# Autodesk Inventor assembly: BaseBotNoMod
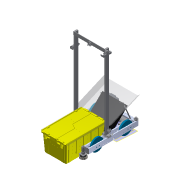
[picture p0: Inventor's stored thumbnail of the model, 180x180]
Saved by Autodesk Inventor 2015 (Build 190159000, 159)
## iProperties
Created: 2015-03-06
Part Number: BaseBotNoMod
Document SubType Name: Assembly
Designer: Kyle
Title: AM14U2 Long FIXED.STEP
Description: STEP AP214
Creation Date: 2015-01-13
Sending System: SolidWorks 2014
Preprocessor: SwSTEP 2.0
Author: Kyle
## Documents named in this file (29)
- C:\Users\Jaden\Desktop\This is why i dont sleep\2015CAD\ReDesign\Project.iam
- C:\Users\Jaden\Desktop\This is why i dont sleep\2015CAD\ReDesign\Imported Components\AM14U2+Long+FIXED\AM14U2 Half Long.iam
- C:\Users\Jaden\Desktop\This is why i dont sleep\2015CAD\ReDesign\Wheel.ipt
- C:\Users\Jaden\Desktop\This is why i dont sleep\2015CAD\ReDesign\Toughbox+Nano+All+Shafts+v2.iam
- C:\Users\Jaden\Desktop\This is why i dont sleep\2015CAD\ReDesign\ControlBoard.ipt
- C:\Users\Jaden\Desktop\This is why i dont sleep\2015CAD\ReDesign\LoadSlide.ipt
- C:\Users\Jaden\Desktop\This is why i dont sleep\2015CAD\ReDesign\FrontSet.ipt
- C:\Users\Jaden\Desktop\This is why i dont sleep\2015CAD\ReDesign\PEG.iam
- C:\Users\Jaden\Desktop\This is why i dont sleep\2015CAD\ReDesign\Slidev2.ipt
- C:\Users\Jaden\Desktop\This is why i dont sleep\2015CAD\ReDesign\YELLOW_TOTEASM_ASM.iam
- C:\Users\Jaden\Desktop\This is why i dont sleep\2015CAD\ReDesign\1x1tbar.ipt
- C:\Users\Jaden\Desktop\This is why i dont sleep\2015CAD\ReDesign\Lift Towers.ipt
- C:\Users\Jaden\Desktop\This is why i dont sleep\2015CAD\ReDesign\motorbracket.ipt
- C:\Users\Jaden\Desktop\This is why i dont sleep\2015CAD\ReDesign\PG188 (1).ipt
- C:\Users\Jaden\Desktop\This is why i dont sleep\2015CAD\ReDesign\4 in HiGrip Wheel.iam
- C:\Users\Jaden\Desktop\This is why i dont sleep\2015CAD\ReDesign\ELEC_Battery_NP18-12B.iam.iam
- C:\Users\Jaden\Desktop\This is why i dont sleep\2015CAD\ReDesign\gyro.ipt
- C:\Users\Jaden\Desktop\This is why i dont sleep\2015CAD\ReDesign\chutebracket.ipt
- C:\Users\Jaden\Desktop\This is why i dont sleep\2015CAD\ReDesign\chutebracketv2.ipt
- C:\Users\Jaden\Desktop\This is why i dont sleep\2015CAD\ReDesign\roller.ipt
- C:\Users\Jaden\Desktop\This is why i dont sleep\2015CAD\ReDesign\rollerbracketer.ipt
- C:\Users\Jaden\Desktop\This is why i dont sleep\2015CAD\ReDesign\armTOP.ipt
- C:\Users\Jaden\Desktop\This is why i dont sleep\2015CAD\ReDesign\collar.ipt
- C:\Users\Jaden\Desktop\This is why i dont sleep\2015CAD\ReDesign\shaft.ipt
- C:\Users\Jaden\Desktop\This is why i dont sleep\2015CAD\ReDesign\pulley.ipt
- C:\Users\Jaden\Desktop\This is why i dont sleep\2015CAD\ReDesign\vertplt.ipt
- C:\Users\Jaden\Desktop\This is why i dont sleep\2015CAD\ReDesign\DualMotor.iam
- C:\Users\Jaden\Desktop\This is why i dont sleep\2015CAD\ReDesign\Spool.iam
- ELEC_Battery_NP18-12B.iam
## Components (62 placed, 28 different names)
1. AM14U2 Half Long_1 [sub-assembly] — Rotational:1, Mate:1, Mate:2, Mate:3, Rotational:3, Mate:6, Angle:2, Mate:10, Mate:18, Mate:19, Mate:32, Flush:2, Angle:9, Angle:10, Angle:11, Mate:99, Mate:100, Mate:101, Mate:107, Mate:108, Mate:127, Mate:128, Mate:129, Mate:187, Mate:193, Mate:194, Flush:16, Angle:15, Mate:201
2. AM14U2 Half Long_2 [sub-assembly] — Rotational:2, Mate:1, Mate:2, Mate:3, Rotational:4, Mate:4, Angle:1, Mate:8, Mate:20, Mate:21, Mate:28, Flush:1, Mate:96, Mate:103, Flush:3, Mate:105, Angle:12
3. Wheel:1 — Rotational:1, Mate:7, Mate:93, Tangent:18
4. Wheel:2 — Rotational:2, Mate:5, Tangent:17
5. Wheel:3 — Rotational:3, Tangent:19
6. Wheel:4 — Rotational:4
7. Toughbox+Nano+All+Shafts+v2:1 [sub-assembly] — Mate:6, Mate:7, Angle:2, Mate:130, Flush:11, Mate:131
8. Toughbox+Nano+All+Shafts+v2:2 [sub-assembly] — Mate:4, Mate:5, Angle:1, Angle:3
9. ControlBoard:1 — Mate:8, Angle:3, Mate:10, Mate:125, Mate:133, Mate:135
10. FrontSet:1 — Mate:18, Mate:19, Mate:113, Mate:115, Mate:116
11. FrontSet:2 — Mate:20, Mate:21, Mate:118, Mate:119, Mate:120
12. PEG:1 [sub-assembly] — Mate:28, Flush:1, Mate:104, Mate:112
13. PEG:2 [sub-assembly] — Mate:32, Flush:2, Mate:102
14. YELLOW_TOTEASM_ASM:1 [sub-assembly] — Tangent:19, Angle:9, Angle:10
15. LoadSlide:1 — Mate:96, Angle:11, Mate:97, Mate:98, Mate:125, Mate:132, Mate:134, Mate:136, Mate:137, Mate:139
16. Slidev2:1 — Mate:97, Mate:98, Mate:99
17. 1x1tbar:1 — Mate:103, Flush:3, Mate:104, Mate:106, Mate:111, Flush:6
18. 1x1tbar:2 — Mate:100, Mate:101, Mate:102, Mate:109, Mate:110, Flush:4, Flush:5
19. Lift Towers:1 — Mate:110, Flush:4, Flush:5, Angle:14, Flush:13, Flush:14, Mate:174, Mate:175, Mate:176, Mate:183, Mate:184
20. 1x1tbar:3 — Mate:105, Mate:106, Angle:12
21. 1x1tbar:5 — Mate:107, Mate:108, Mate:109
22. Lift Towers:2 — Mate:111, Flush:6, Mate:112, Flush:12, Tangent:20, Angle:13, Mate:147, Mate:148, Mate:149
23. motorbracket:1 — Mate:113, Mate:114, Mate:115, Mate:116, Flush:8
24. motorbracket:2 — Mate:118, Mate:119, Mate:120, Mate:121, Flush:10
25. PG188 (1):1 — Mate:114, Mate:117, Flush:7
26. PG188 (1):2 — Mate:121, Mate:122, Flush:9
27. 4 in HiGrip Wheel:1 [sub-assembly] — Mate:117, Flush:7, Flush:8
28. 4 in HiGrip Wheel:2 [sub-assembly] — Mate:122, Flush:9, Flush:10
29. ELEC_Battery_NP18-12B.iam:1 [sub-assembly] — Mate:127, Mate:128, Mate:129
30. gyro:1 — Mate:130, Flush:11, Mate:131
31. chutebracket:1 — Mate:132, Mate:133, Mate:134
32. chutebracket:2 — Mate:135, Mate:136, Mate:137, Mate:138
33. chutebracketv2:1 — Mate:138, Mate:139
34. roller:1 — Flush:12, Tangent:20, Angle:13, Mate:142, Mate:143
35. roller:2 — Angle:14, Flush:13, Flush:14, Mate:144, Mate:145, Mate:146
36. rollerbracketer:1 — Mate:142, Mate:143
37. rollerbracketer:2 — Mate:144, Mate:145, Mate:146
38. armTOP:1 — Mate:147, Mate:148, Mate:149, Mate:156, Mate:159, Mate:160, Mate:163, Mate:165, Mate:172
39. collar:1 — Mate:152, Mate:158
40. shaft:1 — Mate:151, Mate:152, Mate:153, Mate:155, Mate:159, Mate:161
41. pulley:1 — Mate:151, Mate:158, Mate:162
42. collar:2 — Mate:153, Mate:155, Mate:156
43. collar:3 — Mate:160, Mate:161, Mate:162
44. collar:4 — Mate:164, Mate:171, Mate:172, Mate:173
45. shaft:2 — Mate:163, Mate:164, Mate:166, Mate:167, Mate:168, Mate:171, Mate:173
46. pulley:2 — Mate:167, Mate:169, Mate:170
47. collar:5 — Mate:165, Mate:166, Mate:169
48. collar:6 — Mate:168, Mate:170
49. collar:7 — Mate:178, Mate:182, Mate:184
50. shaft:3 — Mate:176, Mate:178, Mate:179, Mate:180, Mate:181, Flush:15, Mate:185
51. pulley:3 — Mate:179, Mate:182, Mate:186
52. vertplt:1 — Mate:174, Mate:175
53. collar:8 — Mate:180, Flush:15, Mate:183
54. collar:9 — Mate:181, Mate:185, Mate:186
55. collar:10 — Mate:188, Mate:192, Mate:193
56. shaft:4 — Mate:187, Mate:188, Mate:189, Mate:190, Mate:191, Mate:192
57. pulley:4 — Mate:191, Mate:195, Mate:196
58. collar:11 — Mate:189, Mate:196
59. collar:12 — Mate:190, Mate:194, Mate:195
60. DualMotor:1 [sub-assembly] — Mate:199, Angle:15, Mate:200, Flush:17
61. 1x1tbar:6 — Flush:16, Mate:199, Mate:201
62. Spool:1 [sub-assembly] — Mate:200, Flush:17
## Relationships (148: Mate 111, Flush 17, Angle 12, RevoluteJoint 4, Tangent 4)
- Rotational:1 [RevoluteJoint] (38.1 mm): AM14U2 Half Long_1 ↔ Wheel:1
- Rotational:2 [RevoluteJoint] (55.88 mm): AM14U2 Half Long_2 ↔ Wheel:2
- Mate:1: AM14U2 Half Long_1 ↔ AM14U2 Half Long_2
- Mate:2: AM14U2 Half Long_1 ↔ AM14U2 Half Long_2
- Mate:3: AM14U2 Half Long_1 ↔ AM14U2 Half Long_2
- Rotational:3 [RevoluteJoint] (57.15 mm): AM14U2 Half Long_1 ↔ Wheel:3
- Rotational:4 [RevoluteJoint] (55.88 mm): AM14U2 Half Long_2 ↔ Wheel:4
- Mate:4: AM14U2 Half Long_2 ↔ Toughbox+Nano+All+Shafts+v2:2
- Mate:5: Wheel:2 ↔ Toughbox+Nano+All+Shafts+v2:2
- Angle:1 (0 deg): AM14U2 Half Long_2 ↔ Toughbox+Nano+All+Shafts+v2:2
- Mate:6: AM14U2 Half Long_1 ↔ Toughbox+Nano+All+Shafts+v2:1
- Mate:7: Wheel:1 ↔ Toughbox+Nano+All+Shafts+v2:1
- Angle:2 (180 deg): AM14U2 Half Long_1 ↔ Toughbox+Nano+All+Shafts+v2:1
- Mate:8: AM14U2 Half Long_2 ↔ ControlBoard:1
- Angle:3 (134.9889 deg): Toughbox+Nano+All+Shafts+v2:2 ↔ ControlBoard:1
- Mate:10: AM14U2 Half Long_1 ↔ ControlBoard:1
- Mate:18: AM14U2 Half Long_1 ↔ FrontSet:1
- Mate:19: AM14U2 Half Long_1 ↔ FrontSet:1
- Mate:20: AM14U2 Half Long_2 ↔ FrontSet:2
- Mate:21: AM14U2 Half Long_2 ↔ FrontSet:2
- Mate:28: AM14U2 Half Long_2 ↔ PEG:1
- Flush:1 (-12.7 mm): AM14U2 Half Long_2 ↔ PEG:1
- Mate:32: AM14U2 Half Long_1 ↔ PEG:2
- Flush:2 (-12.7 mm): AM14U2 Half Long_1 ↔ PEG:2
- Mate:93: Wheel:1
- Angle:7 (0 deg)
- Tangent:17: Wheel:2
- Angle:8 (0 deg)
- Tangent:18: Wheel:1
- Tangent:19: Wheel:3 ↔ YELLOW_TOTEASM_ASM:1
- Angle:9 (179.9087 deg): AM14U2 Half Long_1 ↔ YELLOW_TOTEASM_ASM:1
- Angle:10 (0 deg): AM14U2 Half Long_1 ↔ YELLOW_TOTEASM_ASM:1
- Mate:96 (-63.5 mm): AM14U2 Half Long_2 ↔ LoadSlide:1
- Angle:11 (203.4 deg): AM14U2 Half Long_1 ↔ LoadSlide:1
- Mate:97: LoadSlide:1 ↔ Slidev2:1
- Mate:98: LoadSlide:1 ↔ Slidev2:1
- Mate:99: AM14U2 Half Long_1 ↔ Slidev2:1
- Mate:100: AM14U2 Half Long_1 ↔ 1x1tbar:2
- Mate:101: AM14U2 Half Long_1 ↔ 1x1tbar:2
- Mate:102 (38.1 mm): PEG:2 ↔ 1x1tbar:2
- Mate:103: AM14U2 Half Long_2 ↔ 1x1tbar:1
- Flush:3 (-12.7 mm): AM14U2 Half Long_2 ↔ 1x1tbar:1
- Mate:104 (38.1 mm): PEG:1 ↔ 1x1tbar:1
- Mate:105: AM14U2 Half Long_2 ↔ 1x1tbar:3
- Mate:106: 1x1tbar:1 ↔ 1x1tbar:3
- Angle:12 (0 deg): AM14U2 Half Long_2 ↔ 1x1tbar:3
- Mate:107: AM14U2 Half Long_1 ↔ 1x1tbar:5
- Mate:108: AM14U2 Half Long_1 ↔ 1x1tbar:5
- Mate:109: 1x1tbar:2 ↔ 1x1tbar:5
- Mate:110: 1x1tbar:2 ↔ Lift Towers:1
- Flush:4: 1x1tbar:2 ↔ Lift Towers:1
- Flush:5: 1x1tbar:2 ↔ Lift Towers:1
- Mate:111: 1x1tbar:1 ↔ Lift Towers:2
- Flush:6: 1x1tbar:1 ↔ Lift Towers:2
- Mate:112 (38.1 mm): PEG:1 ↔ Lift Towers:2
- Mate:113: FrontSet:1 ↔ motorbracket:1
- Mate:114: motorbracket:1 ↔ PG188 (1):1
- Mate:115: FrontSet:1 ↔ motorbracket:1
- Mate:116: FrontSet:1 ↔ motorbracket:1
- Mate:117: PG188 (1):1 ↔ 4 in HiGrip Wheel:1
- Flush:7: PG188 (1):1 ↔ 4 in HiGrip Wheel:1
- Flush:8 (-50.8 mm): motorbracket:1 ↔ 4 in HiGrip Wheel:1
- Mate:118: FrontSet:2 ↔ motorbracket:2
- Mate:119: FrontSet:2 ↔ motorbracket:2
- Mate:120: FrontSet:2 ↔ motorbracket:2
- Mate:121: motorbracket:2 ↔ PG188 (1):2
- Mate:122: PG188 (1):2 ↔ 4 in HiGrip Wheel:2
- Flush:9: PG188 (1):2 ↔ 4 in HiGrip Wheel:2
- Flush:10 (-50.8 mm): motorbracket:2 ↔ 4 in HiGrip Wheel:2
- Mate:125: ControlBoard:1 ↔ LoadSlide:1
- Mate:127: AM14U2 Half Long_1 ↔ ELEC_Battery_NP18-12B.iam:1
- Mate:128: AM14U2 Half Long_1 ↔ ELEC_Battery_NP18-12B.iam:1
- Mate:129: AM14U2 Half Long_1 ↔ ELEC_Battery_NP18-12B.iam:1
- Mate:130: Toughbox+Nano+All+Shafts+v2:1 ↔ gyro:1
- Flush:11 (-358.14 mm): Toughbox+Nano+All+Shafts+v2:1 ↔ gyro:1
- Mate:131: Toughbox+Nano+All+Shafts+v2:1 ↔ gyro:1
- Mate:132: LoadSlide:1 ↔ chutebracket:1
- Mate:133: ControlBoard:1 ↔ chutebracket:1
- Mate:134 (190.5 mm): LoadSlide:1 ↔ chutebracket:1
- Mate:135: ControlBoard:1 ↔ chutebracket:2
- Mate:136: LoadSlide:1 ↔ chutebracket:2
- Mate:137 (190.5 mm): LoadSlide:1 ↔ chutebracket:2
- Mate:138: chutebracket:2 ↔ chutebracketv2:1
- Mate:139: LoadSlide:1 ↔ chutebracketv2:1
- Flush:12 (-11.43 mm): Lift Towers:2 ↔ roller:1
- Tangent:20 (-4.445 mm): Lift Towers:2 ↔ roller:1
- Angle:13 (0 deg): Lift Towers:2 ↔ roller:1
- Angle:14 (0 deg): Lift Towers:1 ↔ roller:2
- Flush:13 (-11.43 mm): Lift Towers:1 ↔ roller:2
- Flush:14 (26.67 mm): Lift Towers:1 ↔ roller:2
- Mate:142: roller:1 ↔ rollerbracketer:1
- Mate:143: roller:1 ↔ rollerbracketer:1
- Mate:144: roller:2 ↔ rollerbracketer:2
- Mate:145: roller:2 ↔ rollerbracketer:2
- Mate:146: roller:2 ↔ rollerbracketer:2
- Mate:147: Lift Towers:2 ↔ armTOP:1
- Mate:148: Lift Towers:2 ↔ armTOP:1
- Mate:149: Lift Towers:2 ↔ armTOP:1
- Mate:151: shaft:1 ↔ pulley:1
- Mate:152: collar:1 ↔ shaft:1
- Mate:153: shaft:1 ↔ collar:2
- Mate:155: shaft:1 ↔ collar:2
- Mate:156: armTOP:1 ↔ collar:2
- Mate:158: collar:1 ↔ pulley:1
- Mate:159: armTOP:1 ↔ shaft:1
- Mate:160: armTOP:1 ↔ collar:3
- Mate:161: shaft:1 ↔ collar:3
- Mate:162: pulley:1 ↔ collar:3
- Mate:163: armTOP:1 ↔ shaft:2
- Mate:164: collar:4 ↔ shaft:2
- Mate:165: armTOP:1 ↔ collar:5
- Mate:166: shaft:2 ↔ collar:5
- Mate:167: shaft:2 ↔ pulley:2
- Mate:168: shaft:2 ↔ collar:6
- Mate:169: pulley:2 ↔ collar:5
- Mate:170: pulley:2 ↔ collar:6
- Mate:171: collar:4 ↔ shaft:2
- Mate:172: armTOP:1 ↔ collar:4
- Mate:173: collar:4 ↔ shaft:2
- Mate:174 (12.7 mm): Lift Towers:1 ↔ vertplt:1
- Mate:175: Lift Towers:1 ↔ vertplt:1
- Mate:176: Lift Towers:1 ↔ shaft:3
- Mate:178: collar:7 ↔ shaft:3
- Mate:179: shaft:3 ↔ pulley:3
- Mate:180: shaft:3 ↔ collar:8
- Mate:181: shaft:3 ↔ collar:9
- Mate:182: collar:7 ↔ pulley:3
- Flush:15: shaft:3 ↔ collar:8
- Mate:183: Lift Towers:1 ↔ collar:8
- Mate:184: Lift Towers:1 ↔ collar:7
- Mate:185: shaft:3 ↔ collar:9
- Mate:186: pulley:3 ↔ collar:9
- Mate:187: AM14U2 Half Long_1 ↔ shaft:4
- Mate:188: collar:10 ↔ shaft:4
- Mate:189: shaft:4 ↔ collar:11
- Mate:190: shaft:4 ↔ collar:12
- Mate:191: shaft:4 ↔ pulley:4
- Mate:192: collar:10 ↔ shaft:4
- Mate:193: AM14U2 Half Long_1 ↔ collar:10
- Mate:194: AM14U2 Half Long_1 ↔ collar:12
- Mate:195: pulley:4 ↔ collar:12
- Mate:196: pulley:4 ↔ collar:11
- Flush:16 (-234.95 mm): AM14U2 Half Long_1 ↔ 1x1tbar:6
- Mate:199: DualMotor:1 ↔ 1x1tbar:6
- Angle:15 (179.9087 deg): AM14U2 Half Long_1 ↔ DualMotor:1
- Mate:200: DualMotor:1 ↔ Spool:1
- Mate:201: AM14U2 Half Long_1 ↔ 1x1tbar:6
- Flush:17 (50.8 mm): DualMotor:1 ↔ Spool:1
